# Autodesk Inventor assembly: Bearing_Down_Assembly
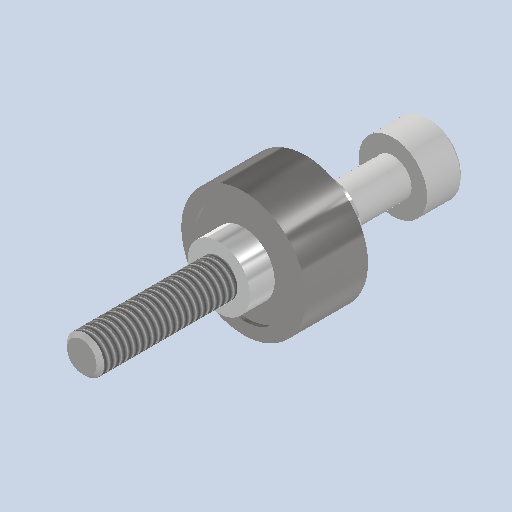
[picture p0: Inventor's stored thumbnail of the model, 512x512]
Saved by Autodesk Inventor 2025.1 (Build 291241020, 241B)
## iProperties
Created: 2024-11-07
Part Number: Bearing_Down_Assembly
Document SubType Name: Assembly
Designer: leon-
Author: leon-
## Documents named in this file (4)
- C:\Users\leon-\OneDrive\Dokumente\Education\Berkeley\Embedded_Systems\Project\CAD_Model\Bearing_Down_Assembly.iam
- C:\Users\leon-\OneDrive\Dokumente\Education\Berkeley\Embedded_Systems\Project\CAD_Model\Purchase_Parts\Bearing_BS69310-5.ipt
- C:\Users\leon-\OneDrive\Dokumente\Education\Berkeley\Embedded_Systems\Project\CAD_Model\Bearing_Distance_Sleeve.ipt
- C:\Users\leon-\OneDrive\Dokumente\Education\Berkeley\Embedded_Systems\Project\CAD_Model\Purchase_Parts\SNSX-M3-25-88.ipt
## Components (4 placed, 3 different names)
1. Bearing_BS69310-5:1 — Mate:1, Mate:2, Mate:3, Mate:4
2. Bearing_Distance_Sleeve:1 — Mate:2, Mate:4, Mate:6
3. Bearing_Distance_Sleeve:2 — Mate:1, Mate:3, Mate:5
4. SNSX-M3-25-88:1 — Mate:5, Mate:6
## Relationships (6: Mate 6)
- Mate:1: Bearing_BS69310-5:1 ↔ Bearing_Distance_Sleeve:2
- Mate:2: Bearing_BS69310-5:1 ↔ Bearing_Distance_Sleeve:1
- Mate:3: Bearing_BS69310-5:1 ↔ Bearing_Distance_Sleeve:2
- Mate:4: Bearing_BS69310-5:1 ↔ Bearing_Distance_Sleeve:1
- Mate:5: Bearing_Distance_Sleeve:2 ↔ SNSX-M3-25-88:1
- Mate:6 (5 mm): Bearing_Distance_Sleeve:1 ↔ SNSX-M3-25-88:1
